# Autodesk Inventor assembly: HandleUnit
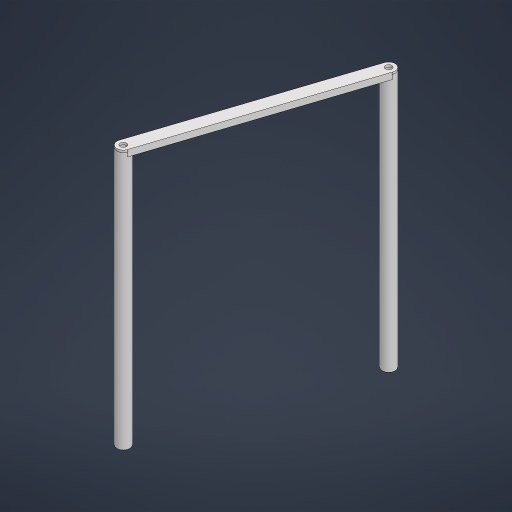
[picture p0: Inventor's stored thumbnail of the model, 512x512]
Saved by Autodesk Inventor 2024.2 (Build 282272000, 272)
## iProperties
Created: 2023-12-28
Part Number: HandleUnit
Document SubType Name: Assembly
Designer: Hanaoka
Author: Hanaoka
## Documents named in this file (3)
- G:\共有ドライブ\reRo\05_個人\hanaoka\inventor\HandleUnit\HandleUnit.iam
- G:\共有ドライブ\reRo\05_個人\hanaoka\inventor\HandleUnit\BaseSpacer_M3.ipt
- G:\共有ドライブ\reRo\05_個人\hanaoka\inventor\HandleUnit\MainBar.ipt
## Components (3 placed, 2 different names)
1. BaseSpacer_M3:1 — 挿入:2
2. BaseSpacer_M3:2 — 挿入:1
3. MainBar:1 — 挿入:1, 挿入:2
## Relationships (2: Insert 2)
- 挿入:1 [Insert]: BaseSpacer_M3:2 ↔ MainBar:1
- 挿入:2 [Insert]: BaseSpacer_M3:1 ↔ MainBar:1
